# Autodesk Inventor assembly: ASY Кассета
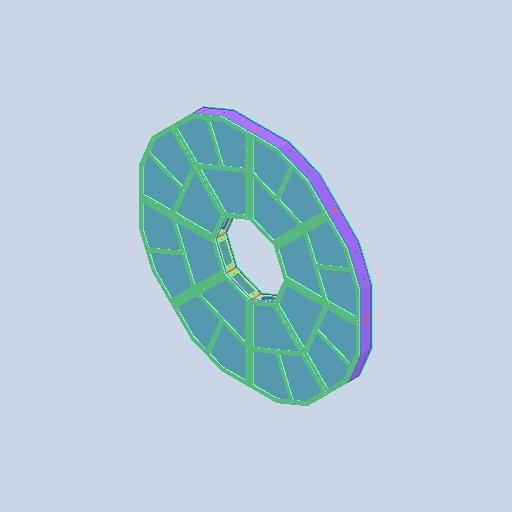
[picture p0: Inventor's stored thumbnail of the model, 512x512]
Saved by Autodesk Inventor 2024.2 (Build 282272000, 272)
## iProperties
Created: 2024-05-05
Part Number: ASY Кассета
Document SubType Name: Assembly
Designer: pokla
Author: pokla
## Documents named in this file (2)
- C:\Users\pokla\Documents\Inventor\ДФО\ДМФ\ДМФ 04.05.24 11-26\ASY ДМФГиД 01011 Кассета.iam
- C:\Users\pokla\Documents\Inventor\ДФО\ДМФ\ДМФ 04.05.24 11-26\ASY Кассета.iam
## Components (8 placed, 1 different names)
1. ASY Кассета:1 [sub-assembly]
2. ASY Кассета:2 [sub-assembly]
3. ASY Кассета:3 [sub-assembly]
4. ASY Кассета:4 [sub-assembly]
5. ASY Кассета:5 [sub-assembly]
6. ASY Кассета:6 [sub-assembly]
7. ASY Кассета:7 [sub-assembly]
8. ASY Кассета:8 [sub-assembly]
## Component patterns: (8 elements, first: ASY Кассета:1)
## Relationships (1: Mate 1)
- [Mate]: ASY Кассета:1
